# Autodesk Inventor assembly: Ring C Assembly
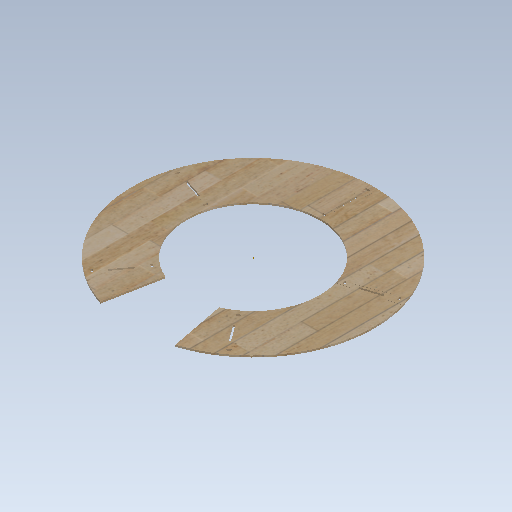
[picture p0: Inventor's stored thumbnail of the model, 512x512]
Saved by Autodesk Inventor 2020 (Build 240168000, 168)
## iProperties
Created: 2020-03-13
Part Number: Ring C Assembly
Document SubType Name: Assembly
Designer: Daniel Wikman
Author: Daniel Wikman
## Documents named in this file (5)
- C:\Users\Dan Wikman\OneDrive\University Life\2020, Semester 1\METR4900 Honours Thesis\Prototype CAD\Ring C Assembly.iam
- C:\Users\Dan Wikman\OneDrive\University Life\2020, Semester 1\METR4900 Honours Thesis\Prototype CAD\Ring C1.ipt
- C:\Users\Dan Wikman\OneDrive\University Life\2020, Semester 1\METR4900 Honours Thesis\Prototype CAD\Ring C2.ipt
- C:\Users\Dan Wikman\OneDrive\University Life\2020, Semester 1\METR4900 Honours Thesis\Prototype CAD\Ring C3.ipt
- C:\Users\Dan Wikman\OneDrive\University Life\2020, Semester 1\METR4900 Honours Thesis\Prototype CAD\Ring C4.ipt
## Components (4 placed, 4 different names)
1. Ring C1:1 — Flush:1, Mate:5, Mate:6
2. Ring C2:1 — Flush:1, Flush:2, Mate:1, Mate:2, Mate:5, Mate:6
3. Ring C3:1 — Flush:2, Flush:3, Mate:1, Mate:2, Mate:3, Mate:4
4. Ring C4:1 — Flush:3, Mate:3, Mate:4
## Relationships (9: Mate 6, Flush 3)
- Flush:1: Ring C1:1 ↔ Ring C2:1
- Flush:2: Ring C2:1 ↔ Ring C3:1
- Flush:3: Ring C3:1 ↔ Ring C4:1
- Mate:1: Ring C2:1 ↔ Ring C3:1
- Mate:2: Ring C2:1 ↔ Ring C3:1
- Mate:3: Ring C3:1 ↔ Ring C4:1
- Mate:4: Ring C3:1 ↔ Ring C4:1
- Mate:5: Ring C1:1 ↔ Ring C2:1
- Mate:6: Ring C1:1 ↔ Ring C2:1
